# Autodesk Inventor assembly: chasis
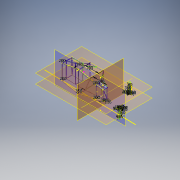
[picture p0: Inventor's stored thumbnail of the model, 180x180]
Saved by Autodesk Inventor 2016 SP1 (Build 200210100, 210)
## iProperties
Created: 2016-06-23
Part Number: chasis
Document SubType Name: Assembly
Designer: asvsf
_SolveAssemblyDoc: Frame Generator Solve Assembly
_Version: 15.0.0
Author: asvsf
## Documents named in this file (5)
- C:\Project\Buggy\chasis.iam
- C:\Project\Buggy\loewr.ipt
- C:\Project\Buggy\chasis\Frame\Frame0001.iam
- C:\Project\Buggy\Suspension\Suspension.iam
- C:\Project\Carv2\suspension_body_001.ipt
## Components (6 placed, 4 different names)
1. lower:1
2. Frame0001:1 [sub-assembly] — Mate:1, Mate:2
3. Suspension:1 [sub-assembly]
4. Suspension:2 [sub-assembly]
5. suspension_body_001:1 — Mate:1
6. suspension_body_001:2 — Mate:2
## Relationships (2: Mate 2)
- Mate:1: Frame0001:1 ↔ suspension_body_001:1
- Mate:2: Frame0001:1 ↔ suspension_body_001:2
